# Autodesk Inventor assembly: in
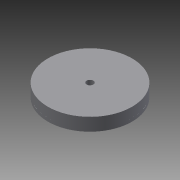
[picture p0: Inventor's stored thumbnail of the model, 180x180]
Saved by Autodesk Inventor 2014 (Build 180170000, 170)
## iProperties
Created: 2013-05-25
Part Number: in
Document SubType Name: Assembly
Designer: Felix
Author: Felix
## Documents named in this file (4)
- C:\Users\Felix\Desktop\Beep\Hardware\Z132053\in.iam
- C:\Users\Felix\Desktop\Beep\Hardware\Z132053\Z53.ipt
- C:\Users\Felix\Desktop\Beep\Hardware\Z132053\inDeckel.ipt
- C:\Users\Felix\Desktop\snap.ipt
## Components (3 placed, 3 different names)
1. Z53:1 — Mate:1, Flush:1
2. inDeckel:1 — Flush:1, Flush:2
3. snap:1 — Mate:3, Flush:2
## Relationships (4: Mate 2, Flush 2)
- Mate:1: Z53:1
- Flush:1: Z53:1 ↔ inDeckel:1
- Mate:3: snap:1
- Flush:2: inDeckel:1 ↔ snap:1
